# Autodesk Inventor assembly: Cheb. korp
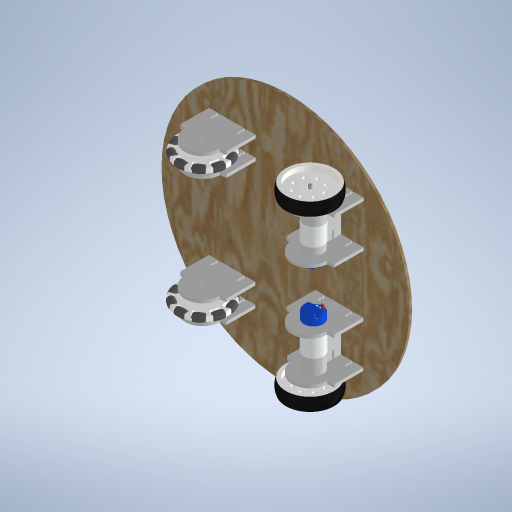
[picture p0: Inventor's stored thumbnail of the model, 512x512]
Saved by Autodesk Inventor 2023.1 (Build 271208000, 208)
## iProperties
Created: 2023-03-13
Part Number: Cheb. korp
Document SubType Name: Assembly
Designer: User
Author: User
## Documents named in this file (16)
- C:\Users\DELL\Desktop\Cheburashka_construction\Cheburashka\korpus\Cheb. korp.iam
- C:\Users\DELL\Desktop\Cheburashka_construction\Cheburashka\korpus\Osn. platform.ipt
- C:\Users\DELL\Desktop\Cheburashka_construction\Cheburashka\korpus\motor1.ipt
- C:\Users\DELL\Desktop\Cheburashka_construction\Cheburashka\korpus\motor2.ipt
- C:\Users\DELL\Desktop\Cheburashka_construction\Cheburashka\korpus\motor3.ipt
- C:\Users\DELL\Desktop\Cheburashka_construction\Cheburashka\korpus\wheel1.ipt
- C:\Users\DELL\Desktop\Cheburashka_construction\Cheburashka\korpus\Импорт\44260_txm torquenado dc motor_MIR2.ipt
- C:\Users\DELL\Desktop\Cheburashka_construction\Cheburashka\korpus\Импорт\36466_txm-4 inch omni wheel.ipt
- C:\Users\DELL\Desktop\Cheburashka_construction\Cheburashka\korpus\Импорт\39055_txm-4 inch wheel_MIR1.ipt
- C:\Users\DELL\Desktop\Cheburashka_construction\Cheburashka\korpus\motor1_MIR3.ipt
- C:\Users\DELL\Desktop\Cheburashka_construction\Cheburashka\korpus\motor2_MIR3.ipt
- C:\Users\DELL\Desktop\Cheburashka_construction\Cheburashka\korpus\motor3_MIR3.ipt
- C:\Users\DELL\Desktop\Cheburashka_construction\Cheburashka\korpus\Импорт\44260_txm torquenado dc motor_MIR2_MIR.ipt
- C:\Users\DELL\Desktop\Cheburashka_construction\Cheburashka\korpus\wheel1_MIR.ipt
- C:\Users\DELL\Desktop\Cheburashka_construction\Cheburashka\korpus\Импорт\36466_txm-4 inch omni wheel_MIR2.ipt
- C:\Users\DELL\Desktop\Cheburashka_construction\Cheburashka\korpus\Импорт\39055_txm-4 inch wheel_MIR1_MIR.ipt
## Components (17 placed, 15 different names)
1. Osn. platform:1 — Совмещение:1, Совмещение:2, Совмещение:3, Совмещение:4, Совмещение:5, Совмещение:6, Совмещение:7, Совмещение:8, Совмещение:9, Совмещение:10, Совмещение:13, Совмещение:14, Совмещение:15, Совмещение:16, Совмещение:17, Совмещение:18
2. motor1:1 — Совмещение:2, Совмещение:3, Совмещение:4
3. motor2:1 — Совмещение:5, Совмещение:6, Совмещение:7
4. motor3:1 — Совмещение:8, Совмещение:9, Совмещение:10, Совмещение:11, Совмещение:12, Совмещение:22
5. 44260_txm torquenado dc motor_MIR2:1 — Совмещение:11, Совмещение:12, Совмещение:21
6. wheel1:1 — Совмещение:13, Совмещение:14, Совмещение:15, Совмещение:19, Совмещение:20
7. wheel1:2 — Совмещение:16, Совмещение:17, Совмещение:18
8. 36466_txm-4 inch omni wheel:1 — Совмещение:19, Совмещение:20
9. 39055_txm-4 inch wheel_MIR1:1 — Совмещение:21, Совмещение:22
10. motor1_MIR3:1
11. motor2_MIR3:1
12. motor3_MIR3:1 — Совмещение:23, Совмещение:24, Совмещение:27
13. 44260_txm torquenado dc motor_MIR2_MIR:1 — Совмещение:23, Совмещение:24, Совмещение:28
14. wheel1_MIR:1 — Совмещение:25, Совмещение:26
15. wheel1_MIR:2
16. 36466_txm-4 inch omni wheel_MIR2:1 — Совмещение:25, Совмещение:26
17. 39055_txm-4 inch wheel_MIR1_MIR:1 — Совмещение:27, Совмещение:28
## Relationships (28: Mate 28)
- Совмещение:1 [Mate]: Osn. platform:1
- Совмещение:2 [Mate]: Osn. platform:1 ↔ motor1:1
- Совмещение:3 [Mate]: Osn. platform:1 ↔ motor1:1
- Совмещение:4 [Mate]: Osn. platform:1 ↔ motor1:1
- Совмещение:5 [Mate]: Osn. platform:1 ↔ motor2:1
- Совмещение:6 [Mate]: Osn. platform:1 ↔ motor2:1
- Совмещение:7 [Mate]: Osn. platform:1 ↔ motor2:1
- Совмещение:8 [Mate]: Osn. platform:1 ↔ motor3:1
- Совмещение:9 [Mate]: Osn. platform:1 ↔ motor3:1
- Совмещение:10 [Mate]: Osn. platform:1 ↔ motor3:1
- Совмещение:11 [Mate]: motor3:1 ↔ 44260_txm torquenado dc motor_MIR2:1
- Совмещение:12 [Mate]: motor3:1 ↔ 44260_txm torquenado dc motor_MIR2:1
- Совмещение:13 [Mate]: Osn. platform:1 ↔ wheel1:1
- Совмещение:14 [Mate]: Osn. platform:1 ↔ wheel1:1
- Совмещение:15 [Mate]: Osn. platform:1 ↔ wheel1:1
- Совмещение:16 [Mate]: Osn. platform:1 ↔ wheel1:2
- Совмещение:17 [Mate]: Osn. platform:1 ↔ wheel1:2
- Совмещение:18 [Mate]: Osn. platform:1 ↔ wheel1:2
- Совмещение:19 [Mate]: wheel1:1 ↔ 36466_txm-4 inch omni wheel:1
- Совмещение:20 [Mate] (10 mm): wheel1:1 ↔ 36466_txm-4 inch omni wheel:1
- Совмещение:21 [Mate]: 44260_txm torquenado dc motor_MIR2:1 ↔ 39055_txm-4 inch wheel_MIR1:1
- Совмещение:22 [Mate] (15 mm): motor3:1 ↔ 39055_txm-4 inch wheel_MIR1:1
- Совмещение:23 [Mate]: motor3_MIR3:1 ↔ 44260_txm torquenado dc motor_MIR2_MIR:1
- Совмещение:24 [Mate]: motor3_MIR3:1 ↔ 44260_txm torquenado dc motor_MIR2_MIR:1
- Совмещение:25 [Mate] (10 mm): wheel1_MIR:1 ↔ 36466_txm-4 inch omni wheel_MIR2:1
- Совмещение:26 [Mate]: wheel1_MIR:1 ↔ 36466_txm-4 inch omni wheel_MIR2:1
- Совмещение:27 [Mate] (15 mm): motor3_MIR3:1 ↔ 39055_txm-4 inch wheel_MIR1_MIR:1
- Совмещение:28 [Mate]: 44260_txm torquenado dc motor_MIR2_MIR:1 ↔ 39055_txm-4 inch wheel_MIR1_MIR:1
